# Autodesk Inventor assembly: Frame
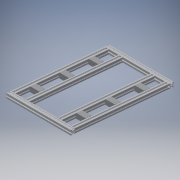
[picture p0: Inventor's stored thumbnail of the model, 180x180]
Saved by Autodesk Inventor 2017 (Build 210142000, 142)
## iProperties
Created: 2017-09-23
Part Number: Frame
Document SubType Name: Assembly
Designer: User
Author: User
## Documents named in this file (4)
- C:\Robotics\CAD\2017-18_CAD\Frame.iam
- C:\Robotics\CAD\COTSParts\Bosch Extrusion\Bosch 20x20 17.5 in 17_18.ipt
- C:\Robotics\CAD\2017-18_CAD\FrameSpacer.ipt
- C:\Robotics\CAD\COTSParts\Bosch Extrusion\Bosch 20x20 11.ipt
## Components (12 placed, 3 different names)
1. Bosch 20x20 17.5 in 17_18:1 — Insert:4, Insert:5, Flush:1, Flush:2, Flush:3, Flush:8
2. Bosch 20x20 17.5 in 17_18:2 — Mate:1, Mate:2, Mate:3, Insert:1, Insert:2, Insert:3, Mate:7, Flush:7
3. FrameSpacer:1 — Mate:1, Insert:1, Insert:4, Flush:1
4. FrameSpacer:2 — Mate:2, Insert:3, Insert:5, Flush:3
5. FrameSpacer:3 — Mate:3, Insert:2, Flush:2
6. Bosch 20x20 17.5 in 17_18:3 — Mate:8, Flush:9
7. Bosch 20x20 17.5 in 17_18:4 — Flush:10, Mate:9, Flush:11, Flush:12
8. FrameSpacer:4
9. FrameSpacer:5
10. FrameSpacer:6
11. Bosch 20x20 11:1 — Mate:7, Flush:7, Flush:8, Mate:8, Flush:9, Flush:10
12. Bosch 20x20 11:2 — Mate:9, Flush:11, Flush:12
## Relationships (31: Flush 12, Insert 10, Mate 9)
- Mate:1: Bosch 20x20 17.5 in 17_18:2 ↔ FrameSpacer:1
- Mate:2: Bosch 20x20 17.5 in 17_18:2 ↔ FrameSpacer:2
- Mate:3: Bosch 20x20 17.5 in 17_18:2 ↔ FrameSpacer:3
- Insert:1: Bosch 20x20 17.5 in 17_18:2 ↔ FrameSpacer:1
- Insert:2: Bosch 20x20 17.5 in 17_18:2 ↔ FrameSpacer:3
- Insert:3: Bosch 20x20 17.5 in 17_18:2 ↔ FrameSpacer:2
- Insert:4: Bosch 20x20 17.5 in 17_18:1 ↔ FrameSpacer:1
- Insert:5: Bosch 20x20 17.5 in 17_18:1 ↔ FrameSpacer:2
- Flush:1: Bosch 20x20 17.5 in 17_18:1 ↔ FrameSpacer:1
- Flush:2: Bosch 20x20 17.5 in 17_18:1 ↔ FrameSpacer:3
- Flush:3: Bosch 20x20 17.5 in 17_18:1 ↔ FrameSpacer:2
- [Mate]: Bosch 20x20 17.5 in 17_18:4 ↔ FrameSpacer:4
- [Mate]: Bosch 20x20 17.5 in 17_18:4 ↔ FrameSpacer:5
- [Mate]: Bosch 20x20 17.5 in 17_18:4 ↔ FrameSpacer:6
- [Insert]: Bosch 20x20 17.5 in 17_18:4 ↔ FrameSpacer:4
- [Insert]: Bosch 20x20 17.5 in 17_18:4 ↔ FrameSpacer:6
- [Insert]: Bosch 20x20 17.5 in 17_18:4 ↔ FrameSpacer:5
- [Insert]: Bosch 20x20 17.5 in 17_18:3 ↔ FrameSpacer:4
- [Insert]: Bosch 20x20 17.5 in 17_18:3 ↔ FrameSpacer:5
- [Flush]: Bosch 20x20 17.5 in 17_18:3 ↔ FrameSpacer:4
- [Flush]: Bosch 20x20 17.5 in 17_18:3 ↔ FrameSpacer:6
- [Flush]: Bosch 20x20 17.5 in 17_18:3 ↔ FrameSpacer:5
- Mate:7: Bosch 20x20 17.5 in 17_18:2 ↔ Bosch 20x20 11:1
- Flush:7: Bosch 20x20 17.5 in 17_18:2 ↔ Bosch 20x20 11:1
- Flush:8: Bosch 20x20 17.5 in 17_18:1 ↔ Bosch 20x20 11:1
- Mate:8: Bosch 20x20 17.5 in 17_18:3 ↔ Bosch 20x20 11:1
- Flush:9: Bosch 20x20 17.5 in 17_18:3 ↔ Bosch 20x20 11:1
- Flush:10: Bosch 20x20 17.5 in 17_18:4 ↔ Bosch 20x20 11:1
- Mate:9: Bosch 20x20 17.5 in 17_18:4 ↔ Bosch 20x20 11:2
- Flush:11: Bosch 20x20 17.5 in 17_18:4 ↔ Bosch 20x20 11:2
- Flush:12: Bosch 20x20 17.5 in 17_18:4 ↔ Bosch 20x20 11:2
## Named parameters: d11_d3 = 0 mm, d12_d4 = 0 mm, d13_d5 = 0 mm, d14_d6 = 0 mm, d15_d7 = 0 mm, d16_d8 = 0 mm, d17_d9 = 0 mm, d18_d10 = 0 mm, d19_d0 = 0 mm, d20_d1 = 0 mm, d21_d2 = 0 mm
